# Autodesk Inventor assembly: cast
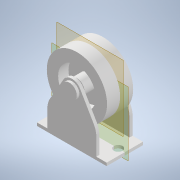
[picture p0: Inventor's stored thumbnail of the model, 180x180]
Saved by Autodesk Inventor 2022 (Build 260153000, 153)
## iProperties
Created: 2022-04-20
Part Number: cast
Document SubType Name: Weldment
Designer: Yazawa
Weld Material: Welded Aluminum-6061
Author: Yazawa
## Documents named in this file (4)
- C:\Users\Yazawa\3D Objects\gigafile-0425-fe8bc7439b67414403b6d7f2877eb22c\cast.iam
- C:\Users\Yazawa\3D Objects\gigafile-0425-fe8bc7439b67414403b6d7f2877eb22c\wheel.ipt
- C:\Users\Yazawa\3D Objects\gigafile-0425-fe8bc7439b67414403b6d7f2877eb22c\castshaft.ipt
- C:\Users\Yazawa\3D Objects\gigafile-0425-fe8bc7439b67414403b6d7f2877eb22c\mounter.ipt
## Components (3 placed, 3 different names)
1. wheel:1 — メイト:1, メイト:3, メイト:4
2. castshaft:1 — メイト:1, メイト:2, メイト:4
3. mounter:1 — メイト:2, メイト:3
## Relationships (4: Mate 4)
- メイト:1 [Mate]: wheel:1 ↔ castshaft:1
- メイト:2 [Mate]: castshaft:1 ↔ mounter:1
- メイト:3 [Mate]: wheel:1 ↔ mounter:1
- メイト:4 [Mate]: wheel:1 ↔ castshaft:1
